# Autodesk Inventor assembly: Hinge
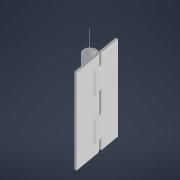
[picture p0: Inventor's stored thumbnail of the model, 180x180]
Saved by Autodesk Inventor 2022 (Build 260153000, 153)
## iProperties
Created: 2021-05-25
Part Number: Hinge
Document SubType Name: Assembly
Designer: Albert L Tomberg
Author: Albert L Tomberg
## Documents named in this file (4)
- C:\Users\Albert L Tomberg\Documents\CAD School\Hinge.iam
- C:\Users\Albert L Tomberg\Documents\CAD School\Poker hinge 1.ipt
- C:\Users\Albert L Tomberg\Documents\CAD School\Poker hinge 2.ipt
- C:\Users\Albert L Tomberg\Documents\CAD School\Poker hinge 3.ipt
## Components (3 placed, 3 different names)
1. Poker hinge 1:1 — Mate:3, Mate:4, Mate:6, Rotational:1
2. Poker hinge 2:1 — Mate:5, Mate:6, Rotational:1
3. Poker hinge 3:1 — Mate:1, Mate:2, Mate:3, Mate:4, Mate:5
## Relationships (7: Mate 6, RevoluteJoint 1)
- Mate:1: Poker hinge 3:1
- Mate:2: Poker hinge 3:1
- Mate:3: Poker hinge 1:1 ↔ Poker hinge 3:1
- Mate:4: Poker hinge 1:1 ↔ Poker hinge 3:1
- Mate:5: Poker hinge 2:1 ↔ Poker hinge 3:1
- Mate:6: Poker hinge 1:1 ↔ Poker hinge 2:1
- Rotational:1 [RevoluteJoint]: Poker hinge 1:1 ↔ Poker hinge 2:1
